# Autodesk Inventor assembly: Assembly_final
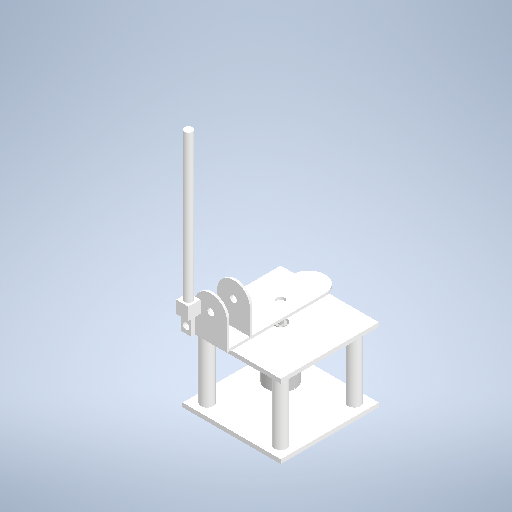
[picture p0: Inventor's stored thumbnail of the model, 512x512]
Saved by Autodesk Inventor 2025.3 (Build 293356000, 356)
## iProperties
Created: 2025-07-22
Part Number: Assembly_final
Document SubType Name: Assembly
Designer: KEVIN
Author: KEVIN
## Documents named in this file (5)
- C:\Users\KEVIN\OneDrive\Documentos\modern_control_project\inverted-pendulum\cad\Assembly_final.iam
- C:\Users\KEVIN\OneDrive\Documentos\modern_control_project\inverted-pendulum\cad\Base_engine.ipt
- C:\Users\KEVIN\OneDrive\Documentos\modern_control_project\inverted-pendulum\cad\Central_base.ipt
- C:\Users\KEVIN\OneDrive\Documentos\modern_control_project\inverted-pendulum\cad\pendulum.ipt
- C:\Users\KEVIN\OneDrive\Documentos\modern_control_project\inverted-pendulum\cad\DC_Motor_GA37RG_12V.ipt
## Components (4 placed, 4 different names)
1. Base_engine:1 — Coincidencia:1, Coincidencia:2
2. Central_base:1 — Coincidencia:2, Coincidencia:3, Coincidencia:4
3. pendulum:1 — Coincidencia:1
4. DC_Motor_GA37RG_12V:1 — Coincidencia:3, Coincidencia:4
## Relationships (4: Mate 4)
- Coincidencia:1 [Mate]: Base_engine:1 ↔ pendulum:1
- Coincidencia:2 [Mate]: Base_engine:1 ↔ Central_base:1
- Coincidencia:3 [Mate]: Central_base:1 ↔ DC_Motor_GA37RG_12V:1
- Coincidencia:4 [Mate]: Central_base:1 ↔ DC_Motor_GA37RG_12V:1
